# Autodesk Inventor assembly: Final_Assembly
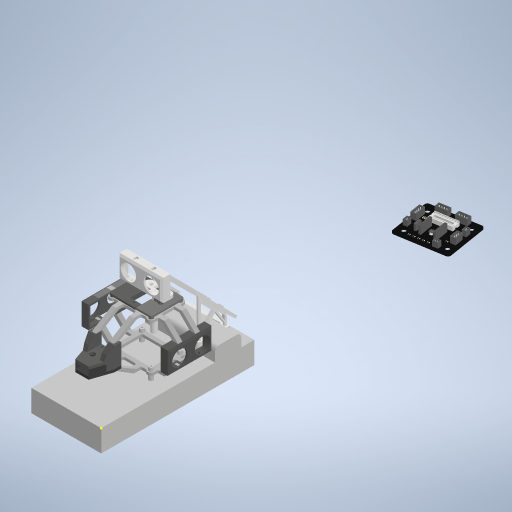
[picture p0: Inventor's stored thumbnail of the model, 512x512]
Saved by Autodesk Inventor 2024 (Build 280153000, 153)
## iProperties
Created: 2024-04-01
Part Number: Final_Assembly
Document SubType Name: Assembly
Designer: ringl
Author: ringl
## Documents named in this file (14)
- C:\Users\ringl\OneDrive\Uni_PC_backup\Y4S2\EE579\Assignment\EE579-Skittles\CAD\Final_Assembly.iam
- C:\Users\ringl\OneDrive\Uni_PC_backup\Y4S2\EE579\Assignment\EE579-Skittles\CAD\CarApproximation.ipt
- C:\Users\ringl\OneDrive\Uni_PC_backup\Y4S2\EE579\Assignment\EE579-Skittles\PCB\EE579_Skittles_pcb\EE579_Skittles_pcb.iam
- C:\Users\ringl\OneDrive\Uni_PC_backup\Y4S2\EE579\Assignment\EE579-Skittles\CAD\TopServoMount.ipt
- C:\Users\ringl\OneDrive\Uni_PC_backup\Y4S2\EE579\Assignment\EE579-Skittles\CAD\Full_Mount.ipt
- C:\Users\ringl\OneDrive\Uni_PC_backup\Y4S2\EE579\Assignment\EE579-Skittles\CAD\UltrasonicSensorMount.ipt
- C:\Users\ringl\OneDrive\Uni_PC_backup\Y4S2\EE579\Assignment\EE579-Skittles\CAD\ServoUltrasonicMount.ipt
- C:\Users\ringl\OneDrive\Uni_PC_backup\Y4S2\EE579\Assignment\EE579-Skittles\CAD\IRMount_bottom.ipt
- C:\Users\ringl\OneDrive\Uni_PC_backup\Y4S2\EE579\Assignment\EE579-Skittles\CAD\IRMount_top.ipt
- C:\Users\ringl\OneDrive\Uni_PC_backup\Y4S2\EE579\Assignment\EE579-Skittles\CAD\ServoFullMountInsert_left.ipt
- C:\Users\ringl\OneDrive\Uni_PC_backup\Y4S2\EE579\Assignment\EE579-Skittles\CAD\ServoFullMountInsert_right.ipt
- C:\Users\ringl\OneDrive\Uni_PC_backup\Y4S2\EE579\Assignment\EE579-Skittles\CAD\ControlPanel\ControlPanel_Bottom.ipt
- C:\Users\ringl\OneDrive\Uni_PC_backup\Y4S2\EE579\Assignment\EE579-Skittles\CAD\ControlPanel\ControlPanel_Middle.ipt
- C:\Users\ringl\OneDrive\Uni_PC_backup\Y4S2\EE579\Assignment\EE579-Skittles\CAD\ControlPanel\ControlPanel_Top.ipt
## Components (17 placed, 13 different names)
1. CarApproximation:1 — Mate:1, Mate:2, Mate:3, Flush:3
2. EE579_Skittles_pcb:1 [sub-assembly] — Mate:1
3. TopServoMount:1
4. Full_Mount:1 — Mate:2, Mate:3, Mate:4, Mate:5, Mate:6, Mate:7, Mate:8, Mate:9, Mate:20, Mate:21, Mate:22
5. UltrasonicSensorMount:1 — Mate:4, Mate:5, Mate:6
6. UltrasonicSensorMount:2 — Mate:7, Mate:8, Mate:9, Mate:16, Mate:17
7. ServoUltrasonicMount:1 — Mate:12, Mate:13, Mate:14
8. UltrasonicSensorMount:4 — Mate:12, Mate:13, Mate:14
9. Full_Mount:2 — Mate:16, Mate:17, Mate:24, Mate:25
10. IRMount_bottom:1 — Mate:20, Mate:21, Mate:22, Mate:23, Flush:1, Flush:2
11. IRMount_top:1 — Mate:23, Flush:1, Flush:2
12. ServoFullMountInsert_left:1 — Mate:24
13. ServoFullMountInsert_right:1 — Mate:25
14. ControlPanel_Bottom:1 — Mate:26, Mate:27, Mate:28, Mate:29
15. ControlPanel_Middle:1 — Mate:26, Mate:27, Mate:30
16. ControlPanel_Middle:2 — Mate:28, Mate:29
17. ControlPanel_Top:1 — Mate:30, Flush:3
## Relationships (28: Mate 25, Flush 3)
- Mate:1 (10 mm): CarApproximation:1 ↔ EE579_Skittles_pcb:1
- Mate:2: CarApproximation:1 ↔ Full_Mount:1
- Mate:3: CarApproximation:1 ↔ Full_Mount:1
- Mate:4 (0.1 mm): Full_Mount:1 ↔ UltrasonicSensorMount:1
- Mate:5: Full_Mount:1 ↔ UltrasonicSensorMount:1
- Mate:6: Full_Mount:1 ↔ UltrasonicSensorMount:1
- Mate:7: Full_Mount:1 ↔ UltrasonicSensorMount:2
- Mate:8 (0.1 mm): Full_Mount:1 ↔ UltrasonicSensorMount:2
- Mate:9: Full_Mount:1 ↔ UltrasonicSensorMount:2
- Mate:12: ServoUltrasonicMount:1 ↔ UltrasonicSensorMount:4
- Mate:13: ServoUltrasonicMount:1 ↔ UltrasonicSensorMount:4
- Mate:14 (0.1 mm): ServoUltrasonicMount:1 ↔ UltrasonicSensorMount:4
- Mate:16: UltrasonicSensorMount:2 ↔ Full_Mount:2
- Mate:17 (0.1 mm): UltrasonicSensorMount:2 ↔ Full_Mount:2
- Mate:20: Full_Mount:1 ↔ IRMount_bottom:1
- Mate:21: Full_Mount:1 ↔ IRMount_bottom:1
- Mate:22: Full_Mount:1 ↔ IRMount_bottom:1
- Mate:23: IRMount_bottom:1 ↔ IRMount_top:1
- Flush:1: IRMount_bottom:1 ↔ IRMount_top:1
- Flush:2: IRMount_bottom:1 ↔ IRMount_top:1
- Mate:24: Full_Mount:2 ↔ ServoFullMountInsert_left:1
- Mate:25: Full_Mount:2 ↔ ServoFullMountInsert_right:1
- Mate:26: ControlPanel_Bottom:1 ↔ ControlPanel_Middle:1
- Mate:27: ControlPanel_Bottom:1 ↔ ControlPanel_Middle:1
- Mate:28: ControlPanel_Bottom:1 ↔ ControlPanel_Middle:2
- Mate:29: ControlPanel_Bottom:1 ↔ ControlPanel_Middle:2
- Mate:30: ControlPanel_Middle:1 ↔ ControlPanel_Top:1
- Flush:3 (12.5 mm): CarApproximation:1 ↔ ControlPanel_Top:1
